# Autodesk Inventor assembly: ensemble_moteur
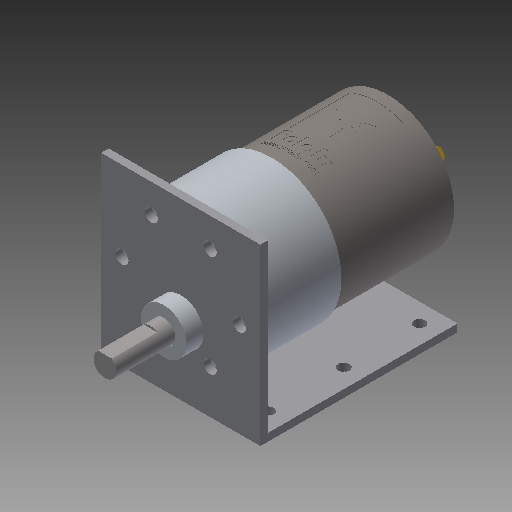
[picture p0: Inventor's stored thumbnail of the model, 512x512]
Saved by Autodesk Inventor 2017 (Build 210142000, 142)
## iProperties
Created: 2016-12-04
Part Number: ensemble_moteur
Document SubType Name: Assembly
Designer: Aegir
Author: Aegir
## Documents named in this file (3)
- C:\Users\franc\Desktop\EsialRobotik\Mecanique\base roulante_v2\conception\ensemble_moteur.iam
- C:\Users\franc\Desktop\EsialRobotik\Mecanique\base roulante_v2\conception\moteur\37d-gearmotor-19-30.ipt
- C:\Users\franc\Desktop\EsialRobotik\Mecanique\base roulante_v2\conception\support_moteur.ipt
## Components (2 placed, 2 different names)
1. 37d-gearmotor-19-30:1 — Affleurement:1
2. support_moteur:1 — Affleurement:1
## Relationships (1: Flush 1)
- Affleurement:1 [Flush]: 37d-gearmotor-19-30:1 ↔ support_moteur:1
